# Autodesk Inventor assembly: Dribbler-3-gears-new
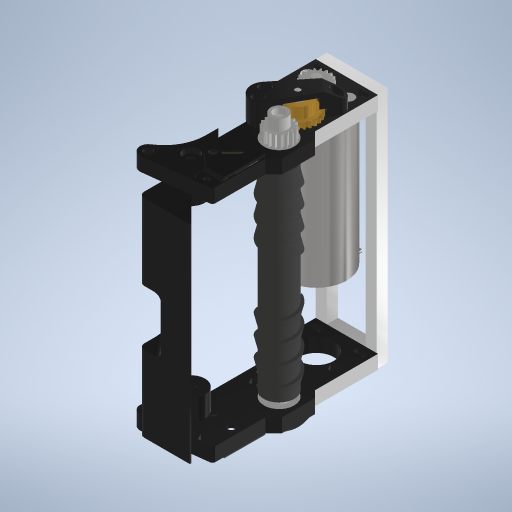
[picture p0: Inventor's stored thumbnail of the model, 512x512]
Saved by Autodesk Inventor 2023 (Build 270158000, 158)
## iProperties
Created: 2021-05-03
Part Number: Dribbler-3-gears-new
Document SubType Name: Assembly
Designer: Acer
Mass: 289.836 g
Surface Area: 495.161 cm^2
Volume: 137.737 cm^3
Density: 2.10428 g/cm^3
Author: Acer
## Documents named in this file (17)
- C:\Users\victo\Documents\MATLAB\CAD\Inventor\first_floor\Dribbler-3-gears\Dribbler-3-gears-new.iam
- C:\Users\victo\Documents\MATLAB\CAD\Inventor\first_floor\Dribbler-3-gears\PartA_3gears_3D.ipt
- C:\Users\victo\Documents\MATLAB\CAD\Inventor\first_floor\Dribbler-3-gears\Kugellager 685-ZZ-C3.ipt
- C:\Users\victo\Documents\MATLAB\CAD\Inventor\first_floor\Dribbler-3-gears\MaxonECmax22-25W.ipt
- C:\Users\victo\Documents\MATLAB\CAD\Inventor\first_floor\Dribbler-3-gears\Eixo.ipt
- C:\Users\victo\Documents\MATLAB\CAD\Inventor\first_floor\Dribbler-3-gears\PartC.ipt
- C:\Users\victo\Documents\MATLAB\CAD\Inventor\first_floor\Dribbler-3-gears\PartB_3gears_3D.ipt
- C:\Users\victo\Documents\MATLAB\CAD\Inventor\first_floor\Dribbler-3-gears\gear_z18_21101800_di3.ipt
- C:\Users\victo\Documents\MATLAB\CAD\Inventor\first_floor\Dribbler-3-gears\gear_z18_21101800(modified).ipt
- C:\Users\victo\Documents\MATLAB\CAD\Inventor\first_floor\Dribbler-3-gears\Middle_Gear.iam
- C:\Users\victo\Documents\MATLAB\CAD\Inventor\first_floor\Dribbler-3-gears\PartD_3D.ipt
- C:\Users\victo\Documents\MATLAB\CAD\Inventor\first_floor\Dribbler-3-gears\Dribblerschnecke.ipt
- C:\Users\victo\Documents\MATLAB\CAD\Inventor\first_floor\Dribbler-3-gears\ChipKicker_v2020_3D.ipt
- C:\Users\victo\Documents\MATLAB\CAD\Inventor\first_floor\Components\IR stuff\PCB Component.iam
- C:\Users\victo\Documents\MATLAB\CAD\Inventor\first_floor\Dribbler-3-gears\PartE.ipt
- C:\Users\victo\Documents\MATLAB\CAD\Inventor\other\Golfball.ipt
- C:\Users\victo\Documents\MATLAB\CAD\Inventor\first_floor\Dribbler-3-gears\PartE_2.ipt
## Components (17 placed, 15 different names)
1. PartA_3gears_3D:1 — Mate:1, Flush:1, Mate:2, Mate:3, Mate:4, Mate:7, Mate:8, Mate:9, Mate:17, Flush:3, Mate:18, Mate:19, Mate:20, Mate:22, Mate:23, Mate:24, Angle:1, Mate:28, Angle:2, Mate:29, Mate:33, Mate:34, Angle:3
2. Kugellager 685-ZZ-C3:1 — Mate:1, Flush:1, Mate:5, Mate:6, Mate:16
3. MaxonECmax22-25W:1 — Mate:2, Mate:3, Mate:4, Mate:13, Mate:14
4. Eixo:1 — Mate:5, Mate:6, Mate:15, Mate:21, Mate:31, Mate:32
5. PartC:1 — Mate:7, Mate:8, Mate:9, Mate:36
6. PartB_3gears_3D:1 — Mate:35, Mate:36, Mate:62, Mate:63
7. Kugellager 685-ZZ-C3:2 — Mate:31, Mate:32, Mate:35
8. Ritzel z=18:1 — Mate:13, Mate:14
9. Ritzel z=18:2 — Mate:15, Mate:16
10. Middle_Gear:1 [sub-assembly] — Mate:17, Flush:3
11. PartD_3D:1 — Mate:18, Mate:19, Mate:20
12. Dribblerschnecke:1 — Mate:21, Mate:22, Tangent:1
13. ChipKicker_v2020_3D:1 — Mate:23, Mate:24, Angle:1, Tangent:2
14. PCB Component:1 [sub-assembly] — Mate:28, Angle:2, Mate:29
15. PartE:1 — Mate:33, Mate:34, Angle:3
16. Golfball:1 — Tangent:1, Tangent:2
17. PartE_2:1 — Mate:62, Mate:63
## Relationships (38: Mate 31, Angle 3, Flush 2, Tangent 2)
- Mate:1: PartA_3gears_3D:1 ↔ Kugellager 685-ZZ-C3:1
- Flush:1: PartA_3gears_3D:1 ↔ Kugellager 685-ZZ-C3:1
- Mate:2: PartA_3gears_3D:1 ↔ MaxonECmax22-25W:1
- Mate:3: PartA_3gears_3D:1 ↔ MaxonECmax22-25W:1
- Mate:4: PartA_3gears_3D:1 ↔ MaxonECmax22-25W:1
- Mate:5: Kugellager 685-ZZ-C3:1 ↔ Eixo:1
- Mate:6: Kugellager 685-ZZ-C3:1 ↔ Eixo:1
- Mate:7: PartA_3gears_3D:1 ↔ PartC:1
- Mate:8: PartA_3gears_3D:1 ↔ PartC:1
- Mate:9: PartA_3gears_3D:1 ↔ PartC:1
- Mate:13: MaxonECmax22-25W:1 ↔ Ritzel z=18:1
- Mate:14: MaxonECmax22-25W:1 ↔ Ritzel z=18:1
- Mate:15: Eixo:1 ↔ Ritzel z=18:2
- Mate:16: Kugellager 685-ZZ-C3:1 ↔ Ritzel z=18:2
- Mate:17: PartA_3gears_3D:1 ↔ Middle_Gear:1
- Flush:3: PartA_3gears_3D:1 ↔ Middle_Gear:1
- Mate:18: PartA_3gears_3D:1 ↔ PartD_3D:1
- Mate:19: PartA_3gears_3D:1 ↔ PartD_3D:1
- Mate:20: PartA_3gears_3D:1 ↔ PartD_3D:1
- Mate:21: Eixo:1 ↔ Dribblerschnecke:1
- Mate:22 (2 mm): PartA_3gears_3D:1 ↔ Dribblerschnecke:1
- Mate:23: PartA_3gears_3D:1 ↔ ChipKicker_v2020_3D:1
- Mate:24 (0.5 mm): PartA_3gears_3D:1 ↔ ChipKicker_v2020_3D:1
- Angle:1 (0 deg): PartA_3gears_3D:1 ↔ ChipKicker_v2020_3D:1
- Mate:28: PartA_3gears_3D:1 ↔ PCB Component:1
- Angle:2 (180 deg): PartA_3gears_3D:1 ↔ PCB Component:1
- Mate:29: PartA_3gears_3D:1 ↔ PCB Component:1
- Mate:31: Eixo:1 ↔ Kugellager 685-ZZ-C3:2
- Mate:32: Eixo:1 ↔ Kugellager 685-ZZ-C3:2
- Mate:33: PartA_3gears_3D:1 ↔ PartE:1
- Mate:34: PartA_3gears_3D:1 ↔ PartE:1
- Angle:3 (0 deg): PartA_3gears_3D:1 ↔ PartE:1
- Mate:35: PartB_3gears_3D:1 ↔ Kugellager 685-ZZ-C3:2
- Mate:36: PartC:1 ↔ PartB_3gears_3D:1
- Tangent:1: Dribblerschnecke:1 ↔ Golfball:1
- Tangent:2: ChipKicker_v2020_3D:1 ↔ Golfball:1
- Mate:62: PartB_3gears_3D:1 ↔ PartE_2:1
- Mate:63: PartB_3gears_3D:1 ↔ PartE_2:1
